# Autodesk Inventor assembly: Последняя ступенька
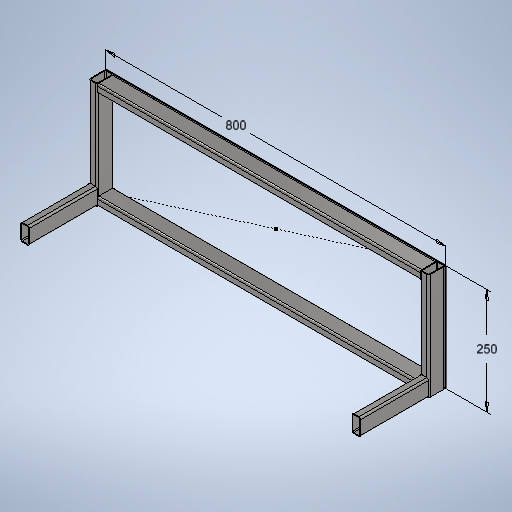
[picture p0: Inventor's stored thumbnail of the model, 512x512]
Saved by Autodesk Inventor 2025 (Build 290162010, 162A)
## iProperties
Created: 2024-09-17
Part Number: Последняя ступенька
Document SubType Name: Assembly
Designer: pokla
_SolveAssemblyDoc: Frame Generator Solve Assembly
_Version: 25.0.0
Author: pokla
## Documents named in this file (4)
- C:\Users\pokla\Documents\Inventor\BSH_Beshkino_bio_tank\Последняя ступенька.iam
- C:\Users\pokla\Documents\Inventor\BSH_Beshkino_bio_tank\Скетч посл. ступ.ipt
- C:\Users\pokla\Documents\Inventor\BSH_Beshkino_bio_tank\Последняя ступенька\Frame\Frame 1726593581865.iam
- C:\Users\pokla\Documents\Inventor\BSH_Beshkino_bio_tank\ISO 4019 - 40x20x2 - 160.ipt
## Components (4 placed, 3 different names)
1. Скетч посл. ступ:1
2. Frame 1726593581865:1 [sub-assembly] — Rigid:1, Rigid:2
3. ISO 4019 - 40x20x2 - 160:1 — Rigid:1
4. ISO 4019 - 40x20x2 - 160:2 — Rigid:2
## Relationships (2: WeldJoint 2)
- Rigid:1 [WeldJoint]: Frame 1726593581865:1 ↔ ISO 4019 - 40x20x2 - 160:1
- Rigid:2 [WeldJoint]: Frame 1726593581865:1 ↔ ISO 4019 - 40x20x2 - 160:2
